# Autodesk Inventor assembly: 組合2
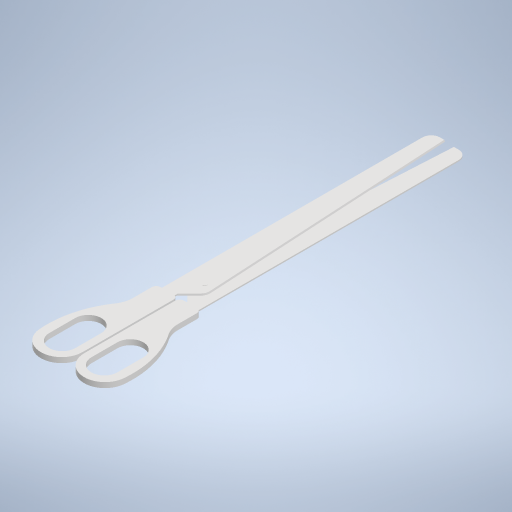
[picture p0: Inventor's stored thumbnail of the model, 512x512]
Saved by Autodesk Inventor 2024.2 (Build 282272000, 272)
## iProperties
Created: 2024-05-16
Part Number: 組合2
Document SubType Name: Assembly
Designer: User
Author: User
## Documents named in this file (4)
- C:\Users\User\OneDrive - 國立中山大學\桌面\創客基礎\0516\組合2.iam
- C:\Users\User\OneDrive - 國立中山大學\桌面\創客基礎\0516\許育菖_刀柄.ipt
- C:\Users\User\OneDrive - 國立中山大學\桌面\創客基礎\0516\許育菖_剪刀握柄.ipt
- C:\Users\User\OneDrive - 國立中山大學\桌面\創客基礎\0516\許育菖_圓柱.ipt
## Components (5 placed, 3 different names)
1. 許育菖_刀柄:1 — 插入:2, 齊平:1, 貼合:2, 貼合:6, 貼合:7
2. 許育菖_刀柄:2 — 插入:1, 齊平:1, 貼合:1, 貼合:3, 貼合:4, 貼合:5
3. 許育菖_剪刀握柄:1 — 貼合:3, 貼合:4, 貼合:5, 齊平:2
4. 許育菖_剪刀握柄:2 — 貼合:6, 貼合:7, 齊平:2
5. 許育菖_圓柱:1 — 插入:1, 插入:2, 貼合:1, 貼合:2
## Relationships (11: Mate 7, Insert 2, Flush 2)
- 插入:1 [Insert] (-1.75 mm): 許育菖_刀柄:2 ↔ 許育菖_圓柱:1
- 插入:2 [Insert] (-0.25 mm): 許育菖_刀柄:1 ↔ 許育菖_圓柱:1
- 齊平:1 [Flush]: 許育菖_刀柄:1 ↔ 許育菖_刀柄:2
- 貼合:1 [Mate]: 許育菖_刀柄:2 ↔ 許育菖_圓柱:1
- 貼合:2 [Mate]: 許育菖_刀柄:1 ↔ 許育菖_圓柱:1
- 貼合:3 [Mate]: 許育菖_刀柄:2 ↔ 許育菖_剪刀握柄:1
- 貼合:4 [Mate]: 許育菖_刀柄:2 ↔ 許育菖_剪刀握柄:1
- 貼合:5 [Mate]: 許育菖_刀柄:2 ↔ 許育菖_剪刀握柄:1
- 貼合:6 [Mate]: 許育菖_刀柄:1 ↔ 許育菖_剪刀握柄:2
- 貼合:7 [Mate]: 許育菖_刀柄:1 ↔ 許育菖_剪刀握柄:2
- 齊平:2 [Flush]: 許育菖_剪刀握柄:1 ↔ 許育菖_剪刀握柄:2
